# Autodesk Inventor assembly: ЛЦМК000002.00.03.00.00.00 Наклонный вариант крепления
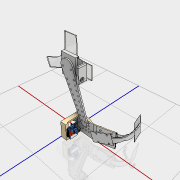
[picture p0: Inventor's stored thumbnail of the model, 180x180]
Saved by Autodesk Inventor 2021.2 (Build 252289000, 289)
## iProperties
Created: 2025-11-10
Part Number: ЛЦМК000002.00.03.00.00.00 Наклонный вариант крепления
Document SubType Name: Assembly
Designer: Захаров
Mass: 54.6297 g
Surface Area: 517.154 cm^2
Volume: 54.6297 cm^3
Density: 1 g/cm^3
Author: Захаров
## Documents named in this file (9)
- C:\Users\User\Documents\CaseARHead1\ЛЦМК000002.00.03.00.00.00 Наклонный вариант крепления.iam
- C:\Users\User\Documents\CaseARHead1\ЛЦМК000002.00.00.00.00.15.ipt
- C:\Users\User\Documents\CaseARHead1\ЛЦМК000002.00.00.00.00.18-01.ipt
- C:\Users\User\Documents\CaseARHead1\ЛЦМК000002.00.00.00.00.06-06.ipt
- C:\Users\User\Documents\CaseARHead1\ЛЦМК000002.00.00.00.00.13 OLED.ipt
- C:\Users\User\Documents\CaseARHead1\ЛЦМК000002.00.00.00.00.14 Фиксатор OLED.ipt
- C:\Users\User\Documents\CaseARHead1\ЛЦМК000002.00.00.00.00.19 мост.ipt
- C:\Users\User\Documents\CaseARHead1\Сборка1.iam
- C:\Users\User\Documents\CaseARHead1\ЛЦМК000002.00.00.00.00.08-01.ipt
## Components (8 placed, 8 different names)
1. ЛЦМК000002.00.00.00.00.15:1 — Совмещение:1, Совмещение:2, Заподлицо:1, Вставка:1, Совмещение:13
2. ЛЦМК000002.00.00.00.00.18-01:1 — Совмещение:1, Совмещение:2, Заподлицо:1, Заподлицо:2, Заподлицо:3, Совмещение:9
3. ЛЦМК000002.00.00.00.00.06-06:1 — Совмещение:3, Угол:1, Совмещение:4, Совмещение:5, Совмещение:6, Совмещение:7, Совмещение:8, Заподлицо:3, Совмещение:9, Совмещение:10, Совмещение:11, Совмещение:12
4. ЛЦМК000002.00.00.00.00.13 OLED:1 — Совмещение:3, Угол:1, Совмещение:7, Совмещение:8
5. ЛЦМК000002.00.00.00.00.14 Фиксатор OLED:1 — Совмещение:4, Совмещение:5, Совмещение:6
6. ЛЦМК000002.00.00.00.00.19 мост:1 — Заподлицо:2, Совмещение:10
7. Сборка1:1 [sub-assembly] — Совмещение:11, Совмещение:12
8. ЛЦМК000002.00.00.00.00.08-01:1 — Вставка:1, Совмещение:13
## Relationships (18: Mate 13, Flush 3, Angle 1, Insert 1)
- Совмещение:1 [Mate]: ЛЦМК000002.00.00.00.00.15:1 ↔ ЛЦМК000002.00.00.00.00.18-01:1
- Совмещение:2 [Mate]: ЛЦМК000002.00.00.00.00.15:1 ↔ ЛЦМК000002.00.00.00.00.18-01:1
- Заподлицо:1 [Flush] (5 mm): ЛЦМК000002.00.00.00.00.15:1 ↔ ЛЦМК000002.00.00.00.00.18-01:1
- Совмещение:3 [Mate]: ЛЦМК000002.00.00.00.00.06-06:1 ↔ ЛЦМК000002.00.00.00.00.13 OLED:1
- Угол:1 [Angle] (-5.5 deg): ЛЦМК000002.00.00.00.00.06-06:1 ↔ ЛЦМК000002.00.00.00.00.13 OLED:1
- Совмещение:4 [Mate]: ЛЦМК000002.00.00.00.00.06-06:1 ↔ ЛЦМК000002.00.00.00.00.14 Фиксатор OLED:1
- Совмещение:5 [Mate]: ЛЦМК000002.00.00.00.00.06-06:1 ↔ ЛЦМК000002.00.00.00.00.14 Фиксатор OLED:1
- Совмещение:6 [Mate]: ЛЦМК000002.00.00.00.00.06-06:1 ↔ ЛЦМК000002.00.00.00.00.14 Фиксатор OLED:1
- Заподлицо:2 [Flush]: ЛЦМК000002.00.00.00.00.18-01:1 ↔ ЛЦМК000002.00.00.00.00.19 мост:1
- Совмещение:7 [Mate]: ЛЦМК000002.00.00.00.00.06-06:1 ↔ ЛЦМК000002.00.00.00.00.13 OLED:1
- Совмещение:8 [Mate]: ЛЦМК000002.00.00.00.00.06-06:1 ↔ ЛЦМК000002.00.00.00.00.13 OLED:1
- Заподлицо:3 [Flush] (30 mm): ЛЦМК000002.00.00.00.00.18-01:1 ↔ ЛЦМК000002.00.00.00.00.06-06:1
- Совмещение:9 [Mate] (70 mm): ЛЦМК000002.00.00.00.00.18-01:1 ↔ ЛЦМК000002.00.00.00.00.06-06:1
- Совмещение:10 [Mate]: ЛЦМК000002.00.00.00.00.06-06:1 ↔ ЛЦМК000002.00.00.00.00.19 мост:1
- Совмещение:11 [Mate]: ЛЦМК000002.00.00.00.00.06-06:1 ↔ Сборка1:1
- Совмещение:12 [Mate]: ЛЦМК000002.00.00.00.00.06-06:1 ↔ Сборка1:1
- Вставка:1 [Insert]: ЛЦМК000002.00.00.00.00.15:1 ↔ ЛЦМК000002.00.00.00.00.08-01:1
- Совмещение:13 [Mate]: ЛЦМК000002.00.00.00.00.15:1 ↔ ЛЦМК000002.00.00.00.00.08-01:1
